# Autodesk Inventor assembly: Shooter P1
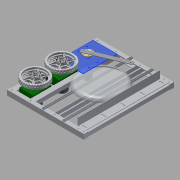
[picture p0: Inventor's stored thumbnail of the model, 180x180]
Saved by Autodesk Inventor 2013 (Build 170138000, 138)
## iProperties
Created: 2013-02-08
Part Number: Shooter P1
Document SubType Name: Assembly
Designer: Naphat
Author: Naphat
## Documents named in this file (8)
- C:\Autodesk\gruntmaster6000-cad\Prototypes\Shooter Firing Pin\Shooter P1.iam
- C:\Autodesk\gruntmaster6000-cad\Shooter\Shooter.iam
- C:\Autodesk\gruntmaster6000-cad\Prototypes\Shooter Firing Pin\Mounting Plate.ipt
- C:\Autodesk\gruntmaster6000-cad\Imported Components\Motors\PG27\PG27.ipt
- C:\Autodesk\gruntmaster6000-cad\Imported Components\Motors\8mm-key-hub\8mm-key-hub.ipt
- C:\Autodesk\gruntmaster6000-cad\Imported Components\Motors\4x4x12 PG-27 Machine Key.ipt
- C:\Autodesk\gruntmaster6000-cad\Prototypes\Shooter Firing Pin\Long Arm.ipt
- C:\Autodesk\gruntmaster6000-cad\Frisbee.ipt
## Components (7 placed, 7 different names)
1. Frisbee:1
2. Shooter:1 [sub-assembly] — Mate:1, Flush:1, Mate:2
3. Mounting Plate:1 — Mate:1, Flush:1, Mate:2, Mate:3, Mate:4
4. PG27:1 — Mate:3, Mate:4, Mate:5, Mate:6, Flush:2, Mate:7, Mate:8
5. 8mm-key-hub:1 — Mate:7, Mate:8, Mate:9, Mate:10, Mate:11
6. 4x4x12 PG-27 Machine Key:1 — Mate:5, Mate:6, Flush:2
7. Long Arm:1 — Mate:9, Mate:10, Mate:11
## Relationships (14: Mate 12, Flush 2)
- Mate:1: Shooter:1 ↔ Mounting Plate:1
- Flush:1: Shooter:1 ↔ Mounting Plate:1
- Mate:2: Shooter:1 ↔ Mounting Plate:1
- Mate:3: Mounting Plate:1 ↔ PG27:1
- Mate:4: Mounting Plate:1 ↔ PG27:1
- Mate:5: PG27:1 ↔ 4x4x12 PG-27 Machine Key:1
- Mate:6: PG27:1 ↔ 4x4x12 PG-27 Machine Key:1
- Flush:2 (-4 mm): PG27:1 ↔ 4x4x12 PG-27 Machine Key:1
- Mate:7: PG27:1 ↔ 8mm-key-hub:1
- Mate:8: PG27:1 ↔ 8mm-key-hub:1
- Mate:9: 8mm-key-hub:1 ↔ Long Arm:1
- Mate:10: 8mm-key-hub:1 ↔ Long Arm:1
- Mate:11: 8mm-key-hub:1 ↔ Long Arm:1
- [Mate]: Frisbee:1 ↔ Shooter:1
